# Autodesk Inventor assembly: Assembly1
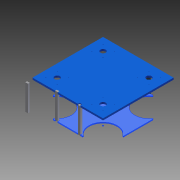
[picture p0: Inventor's stored thumbnail of the model, 180x180]
Saved by Autodesk Inventor 2011 (Build 150239000, 239)
## iProperties
Created: 2011-08-21
Part Number: Assembly1
Document SubType Name: Assembly
Designer: Matthew
Author: Matthew
## Documents named in this file (5)
- C:\Users\Matthew\Documents\matthew_autocad\prlite\base\BASE.iam
- C:\Users\Matthew\Documents\matthew_autocad\prlite\base\base back.ipt
- C:\Users\Matthew\Documents\matthew_autocad\prlite\base\base top.ipt
- C:\Users\Matthew\Documents\matthew_autocad\prlite\base\base bottom.ipt
- C:\Users\Matthew\Documents\matthew_autocad\prlite\base\top-bot connector lame.ipt
## Components (5 placed, 4 different names)
1. base top:1 — Flush:13, Flush:14, Mate:2, Mate:6, Flush:19, Mate:7, Mate:8
2. base bottom:1 — Flush:17, Flush:20, Mate:9
3. base back:1 — Flush:13
4. top-bot connector lame:2 — Flush:14, Mate:2, Flush:17, Mate:7
5. top-bot connector lame:3 — Mate:6, Flush:19, Mate:8, Flush:20, Mate:9
## Relationships (10: Flush 5, Mate 5)
- Flush:13: base top:1 ↔ base back:1
- Flush:14: base top:1 ↔ top-bot connector lame:2
- Mate:2: base top:1 ↔ top-bot connector lame:2
- Flush:17: base bottom:1 ↔ top-bot connector lame:2
- Mate:6: base top:1 ↔ top-bot connector lame:3
- Flush:19: base top:1 ↔ top-bot connector lame:3
- Mate:7: base top:1 ↔ top-bot connector lame:2
- Mate:8: base top:1 ↔ top-bot connector lame:3
- Flush:20: base bottom:1 ↔ top-bot connector lame:3
- Mate:9: base bottom:1 ↔ top-bot connector lame:3
